# Autodesk Inventor assembly: Drive Wheel Assembly V3
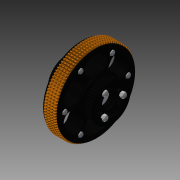
[picture p0: Inventor's stored thumbnail of the model, 180x180]
Saved by Autodesk Inventor 2014 SP1 (Build 180222100, 222)
## iProperties
Created: 2013-01-17
Part Number: Drive Wheel Assembly V3
Document SubType Name: Assembly
Designer: Moses
Mass: 533.698 g
Surface Area: 2049.77 cm^2
Volume: 420.584 cm^3
Density: 1.26895 g/cm^3
Author: Moses
## Documents named in this file (6)
- C:\Users\Moses\Documents\Inventor\Sally Rebuild\Rebuild Sally\Drive Wheel Assembly V3.iam
- C:\Users\Moses\Documents\Inventor\Sally Rebuild\Rebuild Sally\Custom Belt Pulley Hex Hub.ipt
- C:\Users\Moses\Documents\Inventor\Sally Rebuild\Rebuild Sally\DBK_42ToothPulley V2.iam
- C:\Users\Moses\Documents\Inventor\Sally Rebuild\Rebuild Sally\91251A085 (trimmed).ipt
- C:\Users\Moses\Documents\Inventor\Sally Rebuild\Rebuild Sally\91831A011.ipt
- C:\Users\Moses\Documents\Inventor\Sally Rebuild\Rebuild Sally\6Plaction-asm V2.iam
## Components (11 placed, 5 different names)
1. 6Plaction-asm V2:1 [sub-assembly] — Mate:1, Mate:2, Mate:3, Mate:4, Mate:5, Mate:6
2. Custom Belt Pulley Hex Hub:1 — Mate:1, Mate:2, Mate:3, Mate:10, Mate:11, Mate:12
3. Custom Belt Pulley Hex Hub:2 — Mate:4, Mate:5, Mate:6, Mate:7, Mate:8, Mate:9
4. DBK_42ToothPulley V2:1 [sub-assembly] — Mate:7, Mate:8, Mate:9, Insert:1, Insert:2, Insert:3
5. DBK_42ToothPulley V2:2 [sub-assembly] — Mate:10, Mate:11, Mate:12, Insert:4, Insert:5, Insert:6
6. 91251A085 (trimmed):1 — Insert:1
7. 91251A085 (trimmed):2 — Insert:2
8. 91251A085 (trimmed):3 — Insert:3
9. 91831A011:1 — Insert:5
10. 91831A011:2 — Insert:6
11. 91831A011:3 — Insert:4
## Relationships (18: Mate 12, Insert 6)
- Mate:1: 6Plaction-asm V2:1 ↔ Custom Belt Pulley Hex Hub:1
- Mate:2: 6Plaction-asm V2:1 ↔ Custom Belt Pulley Hex Hub:1
- Mate:3: 6Plaction-asm V2:1 ↔ Custom Belt Pulley Hex Hub:1
- Mate:4: 6Plaction-asm V2:1 ↔ Custom Belt Pulley Hex Hub:2
- Mate:5: 6Plaction-asm V2:1 ↔ Custom Belt Pulley Hex Hub:2
- Mate:6: 6Plaction-asm V2:1 ↔ Custom Belt Pulley Hex Hub:2
- Mate:7: Custom Belt Pulley Hex Hub:2 ↔ DBK_42ToothPulley V2:1
- Mate:8: Custom Belt Pulley Hex Hub:2 ↔ DBK_42ToothPulley V2:1
- Mate:9: Custom Belt Pulley Hex Hub:2 ↔ DBK_42ToothPulley V2:1
- Mate:10: Custom Belt Pulley Hex Hub:1 ↔ DBK_42ToothPulley V2:2
- Mate:11: Custom Belt Pulley Hex Hub:1 ↔ DBK_42ToothPulley V2:2
- Mate:12: Custom Belt Pulley Hex Hub:1 ↔ DBK_42ToothPulley V2:2
- Insert:1: DBK_42ToothPulley V2:1 ↔ 91251A085 (trimmed):1
- Insert:2: DBK_42ToothPulley V2:1 ↔ 91251A085 (trimmed):2
- Insert:3: DBK_42ToothPulley V2:1 ↔ 91251A085 (trimmed):3
- Insert:4: DBK_42ToothPulley V2:2 ↔ 91831A011:3
- Insert:5: DBK_42ToothPulley V2:2 ↔ 91831A011:1
- Insert:6: DBK_42ToothPulley V2:2 ↔ 91831A011:2
